# Autodesk Inventor assembly: Assemble
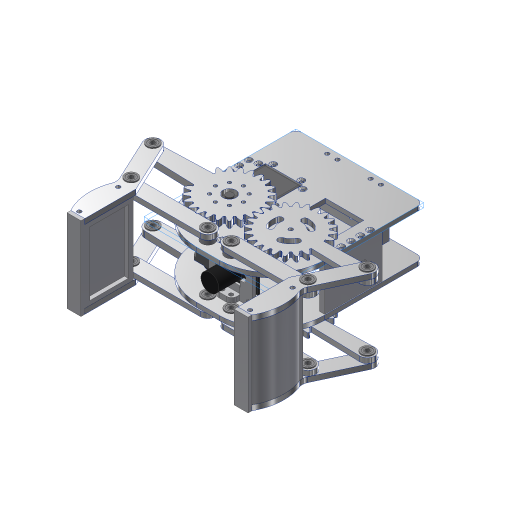
[picture p0: Inventor's stored thumbnail of the model, 512x512]
Saved by Autodesk Inventor 2023.2 (Build 272271000, 271)
## iProperties
Created: 2021-07-28
Part Number: Assemble
Material: 일반
Document SubType Name: Assembly
Designer: user
Mass: 647.33 g
Surface Area: 1523.99 cm^2
Volume: 288.687 cm^3
Density: 2.24233 g/cm^3
Author: user
## Documents named in this file (16)
- C:\Users\BAEK\Desktop\중력보상 프로젝트\Gripper (국방로봇)\Assemble.iam
- C:\Users\BAEK\Desktop\중력보상 프로젝트\Gripper (국방로봇)\RX64_H.ipt
- C:\Users\BAEK\Desktop\중력보상 프로젝트\Gripper (국방로봇)\Box_Back.ipt
- C:\Users\BAEK\Desktop\중력보상 프로젝트\Gripper (국방로봇)\Box_Front.ipt
- C:\Users\BAEK\Desktop\중력보상 프로젝트\Gripper (국방로봇)\Gear_Motor.ipt
- C:\Users\BAEK\Desktop\중력보상 프로젝트\Gripper (국방로봇)\Gear_8T.ipt
- C:\Users\BAEK\Desktop\중력보상 프로젝트\Gripper (국방로봇)\Link.ipt
- C:\Users\BAEK\Desktop\중력보상 프로젝트\Gripper (국방로봇)\Grip_Side_Down.ipt
- C:\Users\BAEK\Desktop\중력보상 프로젝트\Gripper (국방로봇)\Gear_8T_Connect.ipt
- C:\Users\BAEK\Desktop\중력보상 프로젝트\Gripper (국방로봇)\Box_Side.ipt
- C:\Users\BAEK\Desktop\중력보상 프로젝트\Gripper (국방로봇)\Box_Top.ipt
- C:\Users\BAEK\Desktop\중력보상 프로젝트\Gripper (국방로봇)\Camera.iam
- C:\Users\BAEK\Desktop\중력보상 프로젝트\Gripper (국방로봇)\Grip_flange1.ipt
- C:\Users\BAEK\Desktop\중력보상 프로젝트\Gripper (국방로봇)\Grip_flange2.ipt
- C:\Users\BAEK\Desktop\중력보상 프로젝트\Gripper (국방로봇)\FL693ZZ.ipt
- C:\Users\BAEK\Desktop\중력보상 프로젝트\Gripper (국방로봇)\베어링.ipt
## Components (54 placed, 15 different names)
1. RX64_H:1 — 삽입:1, 삽입:2, 삽입:3, 삽입:4, 삽입:121, 삽입:179
2. Box_Back:1 — 삽입:113, 삽입:114, 메이트:3, 메이트:4, 메이트:5, 삽입:180, 삽입:181, 삽입:186, 각도:3, 메이트:40, 메이트:41, 삽입:199
3. Box_Front:1 — 삽입:1, 삽입:2, 삽입:3, 삽입:4, 삽입:69, 삽입:75, 삽입:76, 삽입:77, 삽입:78, 삽입:84, 삽입:85, 삽입:86, 삽입:87, 삽입:88, 삽입:99, 삽입:100, 삽입:101, 삽입:102, 삽입:115, 삽입:116, 메이트:22, 메이트:23, 메이트:24, 메이트:25, 삽입:190, 삽입:191, 메이트:54, 메이트:55, 삽입:203, 각도:4
4. Gear_Motor:1 — 삽입:121, 메이트:34, 메이트:35, 삽입:194
5. Gear_Motor:2 — 삽입:179, 메이트:8, 메이트:9, 삽입:188
6. Link:4 — 메이트:10, 메이트:11, 메이트:12, 메이트:13, 삽입:185, 삽입:187, 각도:3
7. Box_Side:1 — 삽입:69, 삽입:75, 삽입:76, 삽입:77, 삽입:78
8. Box_Side:2 — 삽입:84, 삽입:85, 삽입:86, 삽입:87, 삽입:88
9. Box_Top:1 — 삽입:99, 삽입:100, 삽입:101, 삽입:102
10. Camera:1 [sub-assembly] — 삽입:113, 삽입:114, 삽입:115, 삽입:116
11. FL693ZZ:6 — 메이트:50, 메이트:52
12. Grip_flange2:3 — 삽입:185, 삽입:188, 메이트:14, 메이트:15, 메이트:16, 메이트:17, 삽입:214, 삽입:216
13. FL693ZZ:27 — 메이트:4, 메이트:5
14. FL693ZZ:28 — 메이트:22, 메이트:24
15. FL693ZZ:29 — 메이트:3, 삽입:180
16. 베어링:4 — 삽입:181, 삽입:189
17. Link:5 — 삽입:189, 메이트:18, 메이트:19, 메이트:51, 메이트:53, 삽입:202
18. FL693ZZ:32 — 메이트:14, 메이트:17
19. FL693ZZ:33 — 메이트:15, 메이트:16
20. FL693ZZ:34 — 메이트:10, 메이트:11
21. Grip_flange1:4 — 메이트:36, 메이트:37, 메이트:38, 메이트:39, 삽입:194, 삽입:195, 삽입:215
22. FL693ZZ:35 — 메이트:8, 메이트:9
23. FL693ZZ:36 — 메이트:12, 메이트:13
24. 베어링:5 — 삽입:186, 삽입:187
25. FL693ZZ:38 — 메이트:18, 메이트:19
26. FL693ZZ:39 — 메이트:23, 메이트:25
27. FL693ZZ:41 — 메이트:40, 메이트:41, 삽입:211
28. 베어링:6 — 삽입:190, 삽입:192
29. 베어링:7 — 삽입:191, 삽입:193
30. Link:6 — 삽입:192, 삽입:195
31. FL693ZZ:42
32. FL693ZZ:43
33. Link:7 — 삽입:193, 삽입:206, 각도:4
34. FL693ZZ:44
35. FL693ZZ:45
36. FL693ZZ:47 — 메이트:34, 메이트:35
37. FL693ZZ:48 — 메이트:36, 메이트:39
38. FL693ZZ:49 — 메이트:37, 메이트:38
39. Gear_8T_Connect:2 — 삽입:211
40. 베어링:8 — 삽입:199, 삽입:200
41. Gear_8T:3 — 삽입:200, 메이트:50, 메이트:52, 삽입:201
42. Grip_flange1:5 — 삽입:201, 삽입:202, 삽입:217, 삽입:218
43. FL693ZZ:51
44. FL693ZZ:52
45. FL693ZZ:53 — 메이트:51, 메이트:53
46. FL693ZZ:54 — 메이트:54, 메이트:55
47. Gear_8T:4 — 삽입:204, 메이트:56, 메이트:57, 삽입:205
48. 베어링:9 — 삽입:203, 삽입:204
49. FL693ZZ:55 — 메이트:56, 메이트:57
50. Grip_flange2:4 — 삽입:205, 삽입:206, 삽입:219
51. FL693ZZ:56
52. FL693ZZ:57
53. Grip_Side_Down:5 — 삽입:214, 삽입:215, 삽입:216
54. Grip_Side_Down:6 — 삽입:217, 삽입:218, 삽입:219
## Relationships (105: Insert 52, Mate 51, Angle 2)
- 삽입:1 [Insert]: RX64_H:1 ↔ Box_Front:1
- 삽입:2 [Insert]: RX64_H:1 ↔ Box_Front:1
- 삽입:3 [Insert]: RX64_H:1 ↔ Box_Front:1
- 삽입:4 [Insert]: RX64_H:1 ↔ Box_Front:1
- 삽입:69 [Insert]: Box_Front:1 ↔ Box_Side:1
- 삽입:75 [Insert]: Box_Front:1 ↔ Box_Side:1
- 삽입:76 [Insert]: Box_Front:1 ↔ Box_Side:1
- 삽입:77 [Insert]: Box_Front:1 ↔ Box_Side:1
- 삽입:78 [Insert]: Box_Front:1 ↔ Box_Side:1
- 삽입:84 [Insert]: Box_Front:1 ↔ Box_Side:2
- 삽입:85 [Insert]: Box_Front:1 ↔ Box_Side:2
- 삽입:86 [Insert]: Box_Front:1 ↔ Box_Side:2
- 삽입:87 [Insert]: Box_Front:1 ↔ Box_Side:2
- 삽입:88 [Insert]: Box_Front:1 ↔ Box_Side:2
- 삽입:99 [Insert]: Box_Front:1 ↔ Box_Top:1
- 삽입:100 [Insert]: Box_Front:1 ↔ Box_Top:1
- 삽입:101 [Insert]: Box_Front:1 ↔ Box_Top:1
- 삽입:102 [Insert]: Box_Front:1 ↔ Box_Top:1
- 삽입:113 [Insert] (0.1 mm): Box_Back:1 ↔ Camera:1
- 삽입:114 [Insert] (0.1 mm): Box_Back:1 ↔ Camera:1
- 삽입:115 [Insert] (0.1 mm): Box_Front:1 ↔ Camera:1
- 삽입:116 [Insert] (0.1 mm): Box_Front:1 ↔ Camera:1
- 삽입:121 [Insert]: RX64_H:1 ↔ Gear_Motor:1
- 메이트:3 [Mate]: Box_Back:1 ↔ FL693ZZ:29
- 메이트:4 [Mate]: Box_Back:1 ↔ FL693ZZ:27
- 메이트:5 [Mate]: Box_Back:1 ↔ FL693ZZ:27
- 삽입:179 [Insert]: RX64_H:1 ↔ Gear_Motor:2
- 삽입:180 [Insert]: Box_Back:1 ↔ FL693ZZ:29
- 삽입:181 [Insert]: Box_Back:1 ↔ 베어링:4
- 메이트:8 [Mate]: Gear_Motor:2 ↔ FL693ZZ:35
- 메이트:9 [Mate]: Gear_Motor:2 ↔ FL693ZZ:35
- 메이트:10 [Mate]: Link:4 ↔ FL693ZZ:34
- 메이트:11 [Mate]: Link:4 ↔ FL693ZZ:34
- 메이트:12 [Mate]: Link:4 ↔ FL693ZZ:36
- 메이트:13 [Mate]: Link:4 ↔ FL693ZZ:36
- 삽입:185 [Insert]: Link:4 ↔ Grip_flange2:3
- 삽입:186 [Insert]: Box_Back:1 ↔ 베어링:5
- 삽입:187 [Insert]: Link:4 ↔ 베어링:5
- 삽입:188 [Insert]: Gear_Motor:2 ↔ Grip_flange2:3
- 메이트:14 [Mate]: Grip_flange2:3 ↔ FL693ZZ:32
- 메이트:15 [Mate]: Grip_flange2:3 ↔ FL693ZZ:33
- 메이트:16 [Mate]: Grip_flange2:3 ↔ FL693ZZ:33
- 메이트:17 [Mate]: Grip_flange2:3 ↔ FL693ZZ:32
- 삽입:189 [Insert]: 베어링:4 ↔ Link:5
- 메이트:18 [Mate]: Link:5 ↔ FL693ZZ:38
- 메이트:19 [Mate]: Link:5 ↔ FL693ZZ:38
- 메이트:22 [Mate]: Box_Front:1 ↔ FL693ZZ:28
- 메이트:23 [Mate]: Box_Front:1 ↔ FL693ZZ:39
- 메이트:24 [Mate]: Box_Front:1 ↔ FL693ZZ:28
- 메이트:25 [Mate]: Box_Front:1 ↔ FL693ZZ:39
- 삽입:190 [Insert]: Box_Front:1 ↔ 베어링:6
- 삽입:191 [Insert]: Box_Front:1 ↔ 베어링:7
- [Mate]: Link:6 ↔ FL693ZZ:42
- [Mate]: Link:6 ↔ FL693ZZ:42
- [Mate]: Link:6 ↔ FL693ZZ:43
- [Mate]: Link:6 ↔ FL693ZZ:43
- 삽입:192 [Insert]: 베어링:6 ↔ Link:6
- [Mate]: Link:7 ↔ FL693ZZ:44
- [Mate]: Link:7 ↔ FL693ZZ:44
- [Mate]: Link:7 ↔ FL693ZZ:45
- [Mate]: Link:7 ↔ FL693ZZ:45
- 삽입:193 [Insert]: 베어링:7 ↔ Link:7
- 메이트:34 [Mate]: Gear_Motor:1 ↔ FL693ZZ:47
- 메이트:35 [Mate]: Gear_Motor:1 ↔ FL693ZZ:47
- 메이트:36 [Mate]: Grip_flange1:4 ↔ FL693ZZ:48
- 메이트:37 [Mate]: Grip_flange1:4 ↔ FL693ZZ:49
- 메이트:38 [Mate]: Grip_flange1:4 ↔ FL693ZZ:49
- 메이트:39 [Mate]: Grip_flange1:4 ↔ FL693ZZ:48
- 삽입:194 [Insert]: Gear_Motor:1 ↔ Grip_flange1:4
- 삽입:195 [Insert]: Grip_flange1:4 ↔ Link:6
- 각도:3 [Angle] (0 deg): Box_Back:1 ↔ Link:4
- 메이트:40 [Mate]: Box_Back:1 ↔ FL693ZZ:41
- 메이트:41 [Mate]: Box_Back:1 ↔ FL693ZZ:41
- 삽입:199 [Insert]: Box_Back:1 ↔ 베어링:8
- 삽입:200 [Insert]: 베어링:8 ↔ Gear_8T:3
- [Mate]: Grip_flange1:5 ↔ FL693ZZ:51
- [Mate]: Grip_flange1:5 ↔ FL693ZZ:52
- [Mate]: Grip_flange1:5 ↔ FL693ZZ:52
- [Mate]: Grip_flange1:5 ↔ FL693ZZ:51
- 메이트:50 [Mate]: FL693ZZ:6 ↔ Gear_8T:3
- 메이트:51 [Mate]: Link:5 ↔ FL693ZZ:53
- 메이트:52 [Mate]: FL693ZZ:6 ↔ Gear_8T:3
- 메이트:53 [Mate]: Link:5 ↔ FL693ZZ:53
- 삽입:201 [Insert]: Gear_8T:3 ↔ Grip_flange1:5
- 삽입:202 [Insert]: Link:5 ↔ Grip_flange1:5
- 메이트:54 [Mate]: Box_Front:1 ↔ FL693ZZ:54
- 메이트:55 [Mate]: Box_Front:1 ↔ FL693ZZ:54
- 삽입:203 [Insert]: Box_Front:1 ↔ 베어링:9
- 삽입:204 [Insert]: Gear_8T:4 ↔ 베어링:9
- 메이트:56 [Mate]: Gear_8T:4 ↔ FL693ZZ:55
- 메이트:57 [Mate]: Gear_8T:4 ↔ FL693ZZ:55
- [Mate]: Grip_flange2:4 ↔ FL693ZZ:56
- [Mate]: Grip_flange2:4 ↔ FL693ZZ:57
- [Mate]: Grip_flange2:4 ↔ FL693ZZ:57
- [Mate]: Grip_flange2:4 ↔ FL693ZZ:56
- 삽입:205 [Insert]: Gear_8T:4 ↔ Grip_flange2:4
- 삽입:206 [Insert]: Link:7 ↔ Grip_flange2:4
- 각도:4 [Angle] (0 deg): Box_Front:1 ↔ Link:7
- 삽입:211 [Insert] (0.1 mm): FL693ZZ:41 ↔ Gear_8T_Connect:2
- 삽입:214 [Insert] (0.1 mm): Grip_flange2:3 ↔ Grip_Side_Down:5
- 삽입:215 [Insert] (0.1 mm): Grip_flange1:4 ↔ Grip_Side_Down:5
- 삽입:216 [Insert] (0.1 mm): Grip_flange2:3 ↔ Grip_Side_Down:5
- 삽입:217 [Insert] (0.1 mm): Grip_flange1:5 ↔ Grip_Side_Down:6
- 삽입:218 [Insert] (0.1 mm): Grip_flange1:5 ↔ Grip_Side_Down:6
- 삽입:219 [Insert] (0.1 mm): Grip_flange2:4 ↔ Grip_Side_Down:6
## Named parameters: d291_d267 = 0 mm, d292_d268 = 0 mm, d293_d269 = 0 mm, d294_d270 = 0 mm, d296_d291_d267 = 0 mm, d297_d292_d268 = 0 mm, d298_d293_d269 = 0 mm, d299_d294_d270 = 0 mm, d324_d305 = 0 mm, d325_d306 = 0 mm, d326_d307 = 0 mm, d327_d308 = 0 mm, d341_d276 = 0 mm, d342_d277 = 0 mm, d343_d278 = 0 mm, d344_d279 = 0 mm
